# Autodesk Inventor assembly: Assembly4
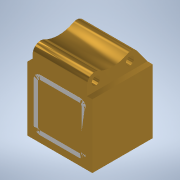
[picture p0: Inventor's stored thumbnail of the model, 180x180]
Saved by Autodesk Inventor 2020 (Build 240168000, 168)
## iProperties
Created: 2022-05-23
Part Number: Assembly4
Document SubType Name: Assembly
Designer: Steven
Author: Steven
## Documents named in this file (3)
- Y:\FPV drone stuff\0 Street League\Frames\PB-Kauri-X\3D prints\35 mm canopy\work in progress prints\session mounts\Assembly4.iam
- Y:\FPV drone stuff\0 Street League\Frames\PB-Kauri-X\3D prints\35 mm canopy\Kauri modular session 5 mount.ipt
- Y:\FPV drone stuff\3d prints\gopro models\session 5.ipt
## Components (2 placed, 2 different names)
1. Kauri modular session 5 mount:1 — Flush:1, Flush:2, Flush:3
2. session 5:1 — Flush:1, Flush:2, Flush:3
## Relationships (3: Flush 3)
- Flush:1: Kauri modular session 5 mount:1 ↔ session 5:1
- Flush:2: Kauri modular session 5 mount:1 ↔ session 5:1
- Flush:3 (1.9 mm): Kauri modular session 5 mount:1 ↔ session 5:1
